# Autodesk Inventor assembly: camera_gimbal.step.STEP.step.STEP
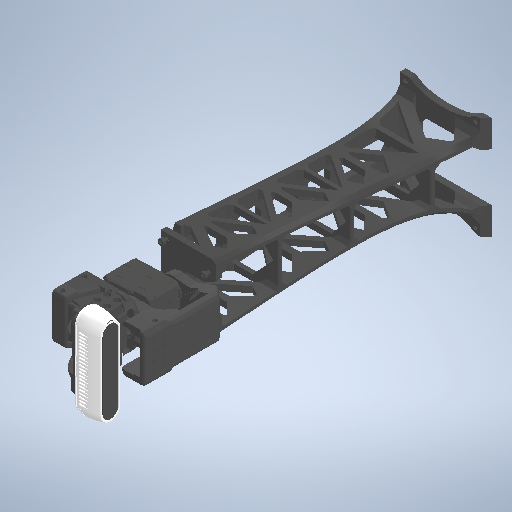
[picture p0: Inventor's stored thumbnail of the model, 512x512]
Saved by Autodesk Inventor 2025.4 (Build 294407000, 407)
## iProperties
Created: 2026-06-01
Part Number: camera_gimbal.step.STEP.step.STEP
Document SubType Name: Assembly
Designer: dalbi
Author: dalbi
## Documents named in this file (8)
- C:\Users\dalbi\OneDrive\바탕 화면\트리보 설계파일\최종 설계 파일(조립시 참고할 파일)\camera_gimbal.step.STEP.step.STEP.iam
- C:\Users\dalbi\OneDrive\바탕 화면\트리보 설계파일\VPK 설계파일(최종본 아님)\root.step.STEP.step.STEP.iam
- C:\Users\dalbi\OneDrive\바탕 화면\트리보 설계파일\VPK 설계파일(최종본 아님)\Wrist_Roll_08c.step.STEP.step.STEP.iam
- C:\Users\dalbi\OneDrive\바탕 화면\트리보 설계파일\VPK 설계파일(최종본 아님)\Gimbal_Pitch_Holder_d435.step.STEP.step.STEP.iam
- C:\Users\dalbi\OneDrive\바탕 화면\트리보 설계파일\VPK 설계파일(최종본 아님)\BSHCS ASME B18.3.1M - M3x0.5 x 12 Steel Grade 2 Plain.step.STEP.step.STEP.ipt
- C:\Users\dalbi\OneDrive\바탕 화면\트리보 설계파일\VPK 설계파일(최종본 아님)\DIN 439-2 - M3 x 0.5 Steel 6 Plain.step.STEP.step.STEP.ipt
- C:\Users\dalbi\OneDrive\바탕 화면\트리보 설계파일\VPK 설계파일(최종본 아님)\Rotation_Pitch_SO101.step.STEP.step.STEP.ipt
- C:\Users\dalbi\OneDrive\바탕 화면\트리보 설계파일\VPK 설계파일(최종본 아님)\SCS215.step.STEP.step.STEP.ipt
## Components (13 placed, 13 different names)
1. root.step.STEP.step.STEP_1 [sub-assembly]
2. Wrist_Roll_08c.step.STEP.step.STEP_1 [sub-assembly]
3. Gimbal_Pitch_Holder_d435.step.STEP.step.STEP_1 [sub-assembly]
4. BSHCS ASME B18.3.1M - M3x0.5 x 12 Steel Grade 2 Plain.step.STEP.step.STEP_1
5. DIN 439-2 - M3 x 0.5 Steel 6 Plain.step.STEP.step.STEP_1
6. BSHCS ASME B18.3.1M - M3x0.5 x 12 Steel Grade 2 Plain.step.STEP.step.STEP_2
7. BSHCS ASME B18.3.1M - M3x0.5 x 12 Steel Grade 2 Plain.step.STEP.step.STEP_3
8. BSHCS ASME B18.3.1M - M3x0.5 x 12 Steel Grade 2 Plain.step.STEP.step.STEP_4
9. DIN 439-2 - M3 x 0.5 Steel 6 Plain.step.STEP.step.STEP_2
10. DIN 439-2 - M3 x 0.5 Steel 6 Plain.step.STEP.step.STEP_3
11. DIN 439-2 - M3 x 0.5 Steel 6 Plain.step.STEP.step.STEP_4
12. Rotation_Pitch_SO101.step.STEP.step.STEP_1 — 메이트:1, 메이트:2
13. SCS215.step.STEP.step.STEP:1 — 메이트:1, 메이트:2
## Relationships (2: Mate 2)
- 메이트:1 [Mate]: Rotation_Pitch_SO101.step.STEP.step.STEP_1 ↔ SCS215.step.STEP.step.STEP:1
- 메이트:2 [Mate]: Rotation_Pitch_SO101.step.STEP.step.STEP_1 ↔ SCS215.step.STEP.step.STEP:1
